# Autodesk Inventor assembly: !Drivebay Left
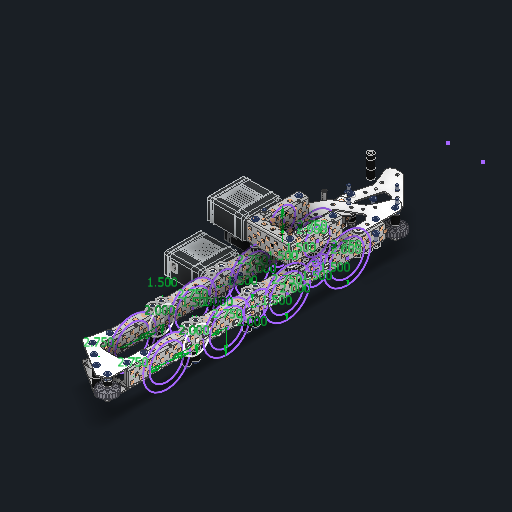
[picture p0: Inventor's stored thumbnail of the model, 512x512]
Saved by Autodesk Inventor 2025.1 (Build 291241000, 241)
## iProperties
Created: 2024-11-11
Part Number: !Drivebay Left
Document SubType Name: Assembly
Designer: avere
Author: avere
## Documents named in this file (6)
- C:\Users\avere\VEX\High Stakes\CAD\V3\Chassis\Drivebay Left\!Drivebay Left.iam
- C:\Users\avere\VEX\High Stakes\CAD\V3\Chassis\Drivebay Left\Structure.iam
- C:\Users\avere\VEX\High Stakes\CAD\ROBOPROS-CAD-Inventor\Electronics\Motors with Screws\SteelM-StarS.iam
- C:\Users\avere\VEX\High Stakes\CAD\ROBOPROS-CAD-Inventor\Electronics\Motors with Screws.iam
- C:\Users\avere\VEX\High Stakes\CAD\V3\Chassis\Drivebay Left\Ring Funnel.iam
- C:\Users\avere\VEX\High Stakes\CAD\V3\Chassis\Drivebay Left\MOGO Funnel Left.iam
## Components (6 placed, 4 different names)
1. Structure:1 [sub-assembly] — Insert:3, Mate:3, Insert:4, Mate:4, Insert:5, Mate:5, Insert:6, Mate:6
2. Ring Funnel:1 [sub-assembly] — Insert:3, Mate:3
3. MOGO Funnel Left:1 [sub-assembly] — Insert:4, Mate:4
4. SteelM-StarS:3 [sub-assembly] — Insert:6, Mate:6
5. SteelM-StarS:1 [sub-assembly] — Insert:5, Mate:5
6. SteelM-StarS:2 [sub-assembly]
## Component patterns: (2 elements, first: SteelM-StarS:1)
## Relationships (8: Insert 4, Mate 4)
- Insert:3: Structure:1 ↔ Ring Funnel:1
- Mate:3: Structure:1 ↔ Ring Funnel:1
- Insert:4: Structure:1 ↔ MOGO Funnel Left:1
- Mate:4: Structure:1 ↔ MOGO Funnel Left:1
- Insert:5: Structure:1 ↔ SteelM-StarS:1
- Mate:5: Structure:1 ↔ SteelM-StarS:1
- Insert:6: Structure:1 ↔ SteelM-StarS:3
- Mate:6: Structure:1 ↔ SteelM-StarS:3
